# Autodesk Inventor assembly: Assembly-omniext
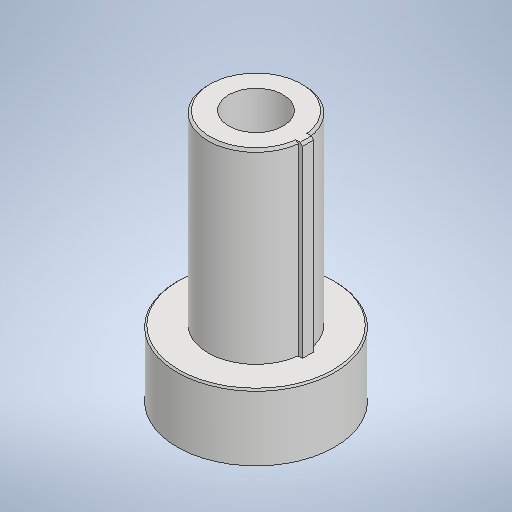
[picture p0: Inventor's stored thumbnail of the model, 512x512]
Saved by Autodesk Inventor 2025.1 (Build 291241000, 241)
## iProperties
Created: 2025-05-08
Part Number: Assembly-omniext
Document SubType Name: Assembly
Designer: User
Author: User
## Documents named in this file (3)
- D:\One Drive\OneDrive - Politeknik Sultan Salahuddin Abdul Aziz Shah\Documents\Inventor\RobosotPSA\Assembly-omniext.iam
- D:\One Drive\OneDrive - Politeknik Sultan Salahuddin Abdul Aziz Shah\Documents\Inventor\RobosotPSA\geared motor brass coupling nut M12 nut 6mm shaft\geared motor brass coupling nut M12 nut 6mm shaft\geared moto.ipt
- D:\One Drive\OneDrive - Politeknik Sultan Salahuddin Abdul Aziz Shah\Documents\Inventor\RobosotPSA\omni_ext.ipt
## Components (2 placed, 2 different names)
1. geared moto:1 — Flush:1, Flush:2
2. omni_ext:1 — Flush:1, Flush:2
## Relationships (2: Flush 2)
- Flush:1: geared moto:1 ↔ omni_ext:1
- Flush:2: geared moto:1 ↔ omni_ext:1
